# Autodesk Inventor assembly: HbIndexFingerForChild
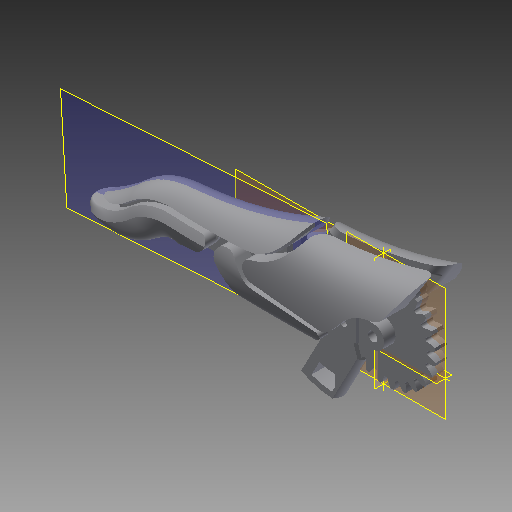
[picture p0: Inventor's stored thumbnail of the model, 512x512]
Saved by Autodesk Inventor 2017 (Build 210142000, 142)
## iProperties
Part Number: HbIndexFingerForChild
Material: 一般
Document SubType Name: Assembly
Designer: sktom
Author: sktom
## Documents named in this file (8)
- D:\OneDrive\CAD\MAJ\hackberry\HACKberry-hardware\3D_69%inlength\Inventor\HbHandForChild\HbIndexFinger01ForChild\HbIndexFinger01ForChild.iam
- D:\OneDrive\CAD\MAJ\hackberry\HACKberry-hardware\3D_69%inlength\Inventor\HbHandForChild\HbIndexFinger01ForChild\HbIndexInputLink02ForChild.ipt
- D:\OneDrive\CAD\MAJ\hackberry\HACKberry-hardware\3D_69%inlength\Inventor\HbHandForChild\HbIndexFinger01ForChild\HbIndexMiddle-DistalPhalanx02ForChild.ipt
- D:\OneDrive\CAD\MAJ\hackberry\HACKberry-hardware\3D_69%inlength\Inventor\HbHandForChild\HbIndexFinger01ForChild\HbIndexCouplerLink02ForChild.ipt
- D:\OneDrive\CAD\MAJ\hackberry\HACKberry-hardware\3D_69%inlength\Inventor\HbHandForChild\HbIndexFinger01ForChild\HbIndexCouplerLinkCover02ForChild.ipt
- D:\OneDrive\CAD\MAJ\hackberry\HACKberry-hardware\3D_69%inlength\Inventor\HbHandForChild\HbIndexFinger01ForChild\HbIndexProximalPhalanx03ForChild.ipt
- D:\OneDrive\CAD\MAJ\hackberry\HACKberry-hardware\3D_69%inlength\Inventor\HbHandForChild\HbIndexFinger01ForChild\HbIndexProximalPhalanxCover02ForChild.ipt
- D:\OneDrive\CAD\MAJ\hackberry\HACKberry-hardware\3D_69%inlength\Inventor\HbHandForChild\HbIndexFinger01ForChild\HbIndexReleaseLever02ForChild.ipt
## Components (7 placed, 7 different names)
1. HbIndexInputLink02ForChild:1 — 挿入:4, 円柱状:1
2. HbIndexMiddle-DistalPhalanx02ForChild:1 — 挿入:1, 挿入:5
3. HbIndexCouplerLink02ForChild:1 — 挿入:1, 挿入:2, 挿入:3, 挿入:4
4. HbIndexCouplerLinkCover02ForChild:1 — 挿入:2, 挿入:3
5. HbIndexProximalPhalanx03ForChild:1 — 挿入:9, 挿入:10
6. HbIndexProximalPhalanxCover02ForChild:1 — 挿入:5, 円柱状:1, 挿入:8, 挿入:9, 挿入:10
7. HbIndexReleaseLever02ForChild:1 — 挿入:8
## Relationships (9: Insert 8, CylindricalJoint 1)
- 挿入:1 [Insert] (0.4 mm): HbIndexMiddle-DistalPhalanx02ForChild:1 ↔ HbIndexCouplerLink02ForChild:1
- 挿入:2 [Insert]: HbIndexCouplerLink02ForChild:1 ↔ HbIndexCouplerLinkCover02ForChild:1
- 挿入:3 [Insert]: HbIndexCouplerLink02ForChild:1 ↔ HbIndexCouplerLinkCover02ForChild:1
- 挿入:4 [Insert] (0.25 mm): HbIndexInputLink02ForChild:1 ↔ HbIndexCouplerLink02ForChild:1
- 挿入:5 [Insert] (0.4 mm): HbIndexMiddle-DistalPhalanx02ForChild:1 ↔ HbIndexProximalPhalanxCover02ForChild:1
- 円柱状:1 [CylindricalJoint]: HbIndexInputLink02ForChild:1 ↔ HbIndexProximalPhalanxCover02ForChild:1
- 挿入:8 [Insert] (0.2 mm): HbIndexProximalPhalanxCover02ForChild:1 ↔ HbIndexReleaseLever02ForChild:1
- 挿入:9 [Insert] (3.5 mm): HbIndexProximalPhalanx03ForChild:1 ↔ HbIndexProximalPhalanxCover02ForChild:1
- 挿入:10 [Insert] (3.5 mm): HbIndexProximalPhalanx03ForChild:1 ↔ HbIndexProximalPhalanxCover02ForChild:1
